# Autodesk Inventor assembly: 6inchMecanumLeft217-2799.20121203
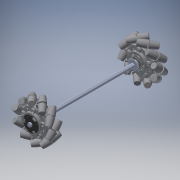
[picture p0: Inventor's stored thumbnail of the model, 180x180]
Saved by Autodesk Inventor 2017 (Build 210142000, 142)
## iProperties
Company: Microsoft
Created: 2012-12-04
Part Number: 6inchMecanumLeft217-2799.20121203
Description: STEP AP203
Document SubType Name: Assembly
Designer: User
Sending System: SolidWorks 2012
Preprocessor: SwSTEP 2.0
Title: 217-2799.20121203.STEP
Author: svradm
Revision Number: ANY
## Documents named in this file (15)
- C:\Robotics\CAD\2017-18_CAD\6_in_mecanum_18_in_axle.iam
- C:\Robotics\CAD\COTSParts\Vex\6inchMecanumLeft217-2799-STEP\217-2799-001 Rev1.ipt
- C:\Robotics\CAD\COTSParts\Vex\6inchMecanumLeft217-2799-STEP\217-2799-002 Rev1.ipt
- C:\Robotics\CAD\COTSParts\Vex\6inchMecanumLeft217-2799-STEP\217-2586-003 Rev2.ipt
- C:\Robotics\CAD\COTSParts\Vex\6inchMecanumLeft217-2799-STEP\217-2586-004 Rev1.ipt
- C:\Robotics\CAD\COTSParts\Vex\6inchMecanumLeft217-2799-STEP\217-2586-007 Rev1.ipt
- C:\Robotics\CAD\COTSParts\Vex\6inchMecanumLeft217-2799-STEP\217-2586-008 Rev1.ipt
- C:\Robotics\CAD\COTSParts\Vex\6inchMecanumLeft217-2799-STEP\NUT-832-NYLOCK.ipt
- C:\Robotics\CAD\COTSParts\Vex\6inchMecanumLeft217-2799-STEP\SCREW-832-1250.ipt
- C:\Robotics\CAD\COTSParts\Vex\6inchMecanumLeft217-2799-STEP\217-2586-005 Rev2.ipt
- C:\Robotics\CAD\COTSParts\Vex\HexAxle.5inchOD217-3309-STEP\HexAxle.5inchOD18inchLength217-3309-STEP.ipt
- C:\Robotics\CAD\COTSParts\Vex\HexBearings.5inchBore217-3875-STEP-20140818\HexBearings.5inchBore217-3875-STEP-20140818.ipt
- C:\Robotics\CAD\COTSParts\Vex\HexSprocket.5inchBore\HexSprocket18t.5inchBore217-3488-STEP\HexSprocket18t.5inchBore217-3488-STEP.ipt
- C:\Robotics\CAD\COTSParts\Vex\VersaHub.5inchBore217-4009-STEP-20140807\VersaHub.5inchBore217-4009-STEP-20140807.ipt
- C:\Robotics\CAD\COTSParts\Vex\6inchMecanumRight217-2586-STEP\6inchMecanumRight217-2586.20121203.ipt
## Components (106 placed, 103 different names)
1. 217-2799-001 Rev1_1 — Insert:2
2. 217-2799-001 Rev1_2 — Insert:1, Mate:1
3. 217-2799-002 Rev1_3
4. 217-2586-003 Rev2_4
5. 217-2586-003 Rev2_5
6. 217-2586-004 Rev1_6
7. 217-2586-004 Rev1_7
8. 217-2586-007 Rev1_8
9. 217-2586-008 Rev1_9
10. NUT-832-NYLOCK_10
11. SCREW-832-1250_11
12. 217-2586-007 Rev1_12
13. 217-2586-007 Rev1_13
14. 217-2586-007 Rev1_14
15. 217-2586-007 Rev1_15
16. 217-2586-007 Rev1_16
17. 217-2586-007 Rev1_17
18. 217-2586-007 Rev1_18
19. 217-2586-007 Rev1_19
20. 217-2586-007 Rev1_20
21. 217-2586-004 Rev1_21
22. 217-2586-004 Rev1_22
23. 217-2586-004 Rev1_23
24. 217-2586-004 Rev1_24
25. 217-2586-004 Rev1_25
26. 217-2586-004 Rev1_26
27. 217-2586-004 Rev1_27
28. 217-2586-004 Rev1_28
29. 217-2586-004 Rev1_29
30. 217-2586-004 Rev1_30
31. 217-2586-004 Rev1_31
32. 217-2586-004 Rev1_32
33. 217-2586-004 Rev1_33
34. 217-2586-004 Rev1_34
35. 217-2586-004 Rev1_35
36. 217-2586-004 Rev1_36
37. 217-2586-004 Rev1_37
38. 217-2586-004 Rev1_38
39. 217-2586-003 Rev2_39
40. 217-2586-003 Rev2_40
41. 217-2586-003 Rev2_41
42. 217-2586-003 Rev2_42
43. 217-2586-003 Rev2_43
44. 217-2586-003 Rev2_44
45. 217-2586-003 Rev2_45
46. 217-2586-003 Rev2_46
47. 217-2586-003 Rev2_47
48. 217-2586-003 Rev2_48
49. 217-2586-003 Rev2_49
50. 217-2586-003 Rev2_50
51. 217-2586-003 Rev2_51
52. 217-2586-003 Rev2_52
53. 217-2586-003 Rev2_53
54. 217-2586-003 Rev2_54
55. 217-2586-003 Rev2_55
56. 217-2586-003 Rev2_56
57. 217-2799-002 Rev1_57
58. 217-2799-002 Rev1_58
59. 217-2799-002 Rev1_59
60. 217-2799-002 Rev1_60
61. 217-2799-002 Rev1_61
62. 217-2799-002 Rev1_62
63. 217-2799-002 Rev1_63
64. 217-2799-002 Rev1_64
65. 217-2799-002 Rev1_65
66. 217-2586-008 Rev1_66
67. 217-2586-008 Rev1_67
68. 217-2586-008 Rev1_68
69. 217-2586-008 Rev1_69
70. 217-2586-008 Rev1_70
71. SCREW-832-1250_71
72. SCREW-832-1250_72
73. SCREW-832-1250_73
74. SCREW-832-1250_74
75. NUT-832-NYLOCK_75
76. NUT-832-NYLOCK_76
77. NUT-832-NYLOCK_77
78. NUT-832-NYLOCK_78
79. 217-2586-005 Rev2_79
80. 217-2586-005 Rev2_80
81. 217-2586-005 Rev2_81
82. 217-2586-005 Rev2_82
83. 217-2586-005 Rev2_83
84. 217-2586-005 Rev2_84
85. 217-2586-005 Rev2_85
86. 217-2586-005 Rev2_86
87. 217-2586-005 Rev2_87
88. 217-2586-005 Rev2_88
89. 217-2586-005 Rev2_89
90. 217-2586-005 Rev2_90
91. 217-2586-005 Rev2_91
92. 217-2586-005 Rev2_92
93. 217-2586-005 Rev2_93
94. 217-2586-005 Rev2_94
95. 217-2586-005 Rev2_95
96. 217-2586-005 Rev2_96
97. 217-2586-005 Rev2_97
98. 217-2586-005 Rev2_98
99. HexAxle.5inchOD18inchLength217-3309-STEP:1 — Mate:3, Mate:4, Mate:5, Flush:2, Mate:7, Mate:9, Mate:10, Flush:3, Mate:11, Mate:13, Mate:14
100. HexBearings.5inchBore217-3875-STEP-20140818:1 — Insert:2, Flush:1, Mate:3, Mate:6
101. HexSprocket18t.5inchBore217-3488-STEP:1 — Mate:4, Mate:5, Mate:6
102. VersaHub.5inchBore217-4009-STEP-20140807:1 — Insert:1, Mate:1, Flush:1, Flush:2, Mate:7
103. 6inchMecanumRight217-2586.20121203:1 — Insert:3, Mate:8, Insert:4
104. HexSprocket18t.5inchBore217-3488-STEP:2 — Mate:12, Mate:13, Mate:14
105. HexBearings.5inchBore217-3875-STEP-20140818:2 — Insert:4, Mate:11, Mate:12
106. VersaHub.5inchBore217-4009-STEP-20140807:2 — Insert:3, Mate:8, Mate:9, Mate:10, Flush:3
## Relationships (20: Mate 13, Insert 4, Flush 3)
- Insert:1: 217-2799-001 Rev1_2 ↔ VersaHub.5inchBore217-4009-STEP-20140807:1
- Mate:1: 217-2799-001 Rev1_2 ↔ VersaHub.5inchBore217-4009-STEP-20140807:1
- Insert:2: 217-2799-001 Rev1_1 ↔ HexBearings.5inchBore217-3875-STEP-20140818:1
- Flush:1: HexBearings.5inchBore217-3875-STEP-20140818:1 ↔ VersaHub.5inchBore217-4009-STEP-20140807:1
- Mate:3: HexAxle.5inchOD18inchLength217-3309-STEP:1 ↔ HexBearings.5inchBore217-3875-STEP-20140818:1
- Mate:4: HexAxle.5inchOD18inchLength217-3309-STEP:1 ↔ HexSprocket18t.5inchBore217-3488-STEP:1
- Mate:5: HexAxle.5inchOD18inchLength217-3309-STEP:1 ↔ HexSprocket18t.5inchBore217-3488-STEP:1
- Mate:6 (3.175 mm): HexBearings.5inchBore217-3875-STEP-20140818:1 ↔ HexSprocket18t.5inchBore217-3488-STEP:1
- Flush:2 (-6.35 mm): HexAxle.5inchOD18inchLength217-3309-STEP:1 ↔ VersaHub.5inchBore217-4009-STEP-20140807:1
- Mate:7: HexAxle.5inchOD18inchLength217-3309-STEP:1 ↔ VersaHub.5inchBore217-4009-STEP-20140807:1
- Insert:3: 6inchMecanumRight217-2586.20121203:1 ↔ VersaHub.5inchBore217-4009-STEP-20140807:2
- Mate:8: 6inchMecanumRight217-2586.20121203:1 ↔ VersaHub.5inchBore217-4009-STEP-20140807:2
- Mate:9: HexAxle.5inchOD18inchLength217-3309-STEP:1 ↔ VersaHub.5inchBore217-4009-STEP-20140807:2
- Mate:10: HexAxle.5inchOD18inchLength217-3309-STEP:1 ↔ VersaHub.5inchBore217-4009-STEP-20140807:2
- Flush:3 (-6.35 mm): HexAxle.5inchOD18inchLength217-3309-STEP:1 ↔ VersaHub.5inchBore217-4009-STEP-20140807:2
- Insert:4: 6inchMecanumRight217-2586.20121203:1 ↔ HexBearings.5inchBore217-3875-STEP-20140818:2
- Mate:11: HexAxle.5inchOD18inchLength217-3309-STEP:1 ↔ HexBearings.5inchBore217-3875-STEP-20140818:2
- Mate:12 (3.175 mm): HexSprocket18t.5inchBore217-3488-STEP:2 ↔ HexBearings.5inchBore217-3875-STEP-20140818:2
- Mate:13: HexAxle.5inchOD18inchLength217-3309-STEP:1 ↔ HexSprocket18t.5inchBore217-3488-STEP:2
- Mate:14: HexAxle.5inchOD18inchLength217-3309-STEP:1 ↔ HexSprocket18t.5inchBore217-3488-STEP:2
